# Autodesk Inventor assembly: Bedienhebel
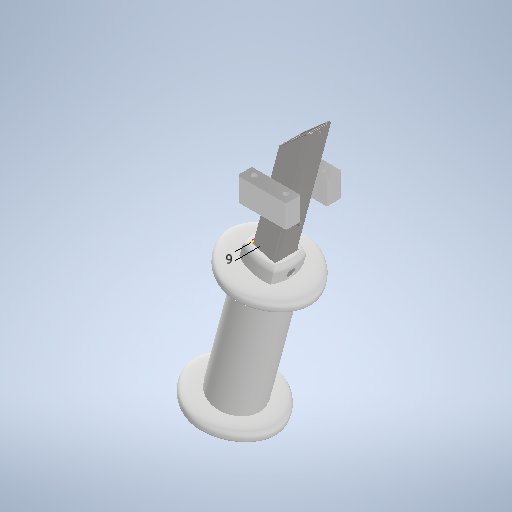
[picture p0: Inventor's stored thumbnail of the model, 512x512]
Saved by Autodesk Inventor 2025 (Build 290162010, 162A)
## iProperties
Created: 2024-11-27
Part Number: Bedienhebel
Document SubType Name: Assembly
Designer: Admin
Author: Admin
## Documents named in this file (11)
- C:\Users\Admin\GIT\HDVKBM\CAD\Krandemonstrator\Bedienhebel.iam
- C:\Users\Admin\GIT\HDVKBM\CAD\Krandemonstrator\HebelhalterBlock.ipt
- C:\Users\Admin\GIT\HDVKBM\CAD\Krandemonstrator\HebelhalterBlockBlind.ipt
- C:\Users\Admin\GIT\HDVKBM\CAD\Krandemonstrator\ISO 12633-2 - 20x20x2 - 200.ipt
- C:\Users\Admin\Documents\Inventor\Content Center Files\R2025\de-DE\DIN 7991(2)\DIN 7991 - M4x40.ipt
- C:\Users\Admin\Documents\Inventor\Content Center Files\R2025\de-DE\AS 1237 (2.1)\AS 1237 - 4.ipt
- C:\Users\Admin\GIT\HDVKBM\CAD\Krandemonstrator\Lagerhülse 6x4x0.ipt
- C:\Users\Admin\GIT\HDVKBM\CAD\Krandemonstrator\knaufErgo.ipt
- C:\Users\Admin\Documents\Inventor\Content Center Files\R2025\de-DE\DIN 7991(2)\DIN 7991 - M3x30.ipt
- C:\Users\Admin\GIT\HDVKBM\CAD\Krandemonstrator\M3 Haken 40mm.ipt
- C:\Users\Admin\Documents\Inventor\Content Center Files\R2025\de-DE\DIN 934\DIN 934 - M3 x 0,5.ipt
## Components (11 placed, 10 different names)
1. HebelhalterBlock:1 — Passend:5, Starr:3, Starr:5
2. HebelhalterBlockBlind:1 — Starr:4, Starr:5, Drehbar:1
3. DIN 7991 M4x40:1 — Passend:5
4. ISO 12633-2 - 20x20x2 - 200:1 — Drehbar:1, Drehbar:2, Verschiebbar:1, Zylindrisch:1, Starr:7, Einfügen:1
5. AS 1237 (2.1) 4:1 — Starr:4
6. AS 1237 (2.1) 4:2 — Starr:3
7. Lagerhülse 6x4x0:1 — Drehbar:2
8. knaufErgo:1 — Starr:6, Verschiebbar:1
9. DIN 7991 M3x30:1 — Starr:6, Zylindrisch:1
10. M3 Haken 40mm:1 — Starr:7
11. DIN 934 - ersetzt durch DIN EN 24032/28673/28674 M3:1 — Einfügen:1
## Relationships (11: WeldJoint 5, RevoluteJoint 2, Mate 1, TranslationJoint 1, CylindricalJoint 1, Insert 1)
- Passend:5 [Mate]: HebelhalterBlock:1 ↔ DIN 7991 M4x40:1
- Starr:3 [WeldJoint]: HebelhalterBlock:1 ↔ AS 1237 (2.1) 4:2
- Drehbar:1 [RevoluteJoint] (1 mm): HebelhalterBlockBlind:1 ↔ ISO 12633-2 - 20x20x2 - 200:1
- Starr:4 [WeldJoint]: HebelhalterBlockBlind:1 ↔ AS 1237 (2.1) 4:1
- Starr:5 [WeldJoint] (-22 mm): HebelhalterBlock:1 ↔ HebelhalterBlockBlind:1
- Drehbar:2 [RevoluteJoint]: ISO 12633-2 - 20x20x2 - 200:1 ↔ Lagerhülse 6x4x0:1
- Starr:6 [WeldJoint]: knaufErgo:1 ↔ DIN 7991 M3x30:1
- Verschiebbar:1 [TranslationJoint]: ISO 12633-2 - 20x20x2 - 200:1 ↔ knaufErgo:1
- Zylindrisch:1 [CylindricalJoint]: ISO 12633-2 - 20x20x2 - 200:1 ↔ DIN 7991 M3x30:1
- Starr:7 [WeldJoint]: ISO 12633-2 - 20x20x2 - 200:1 ↔ M3 Haken 40mm:1
- Einfügen:1 [Insert]: ISO 12633-2 - 20x20x2 - 200:1 ↔ DIN 934 - ersetzt durch DIN EN 24032/28673/28674 M3:1
